# Autodesk Inventor assembly: FT7635M_Servo assembly_with T_BAR
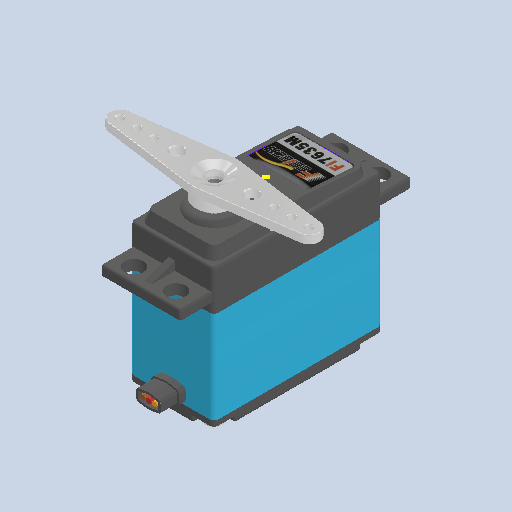
[picture p0: Inventor's stored thumbnail of the model, 512x512]
Saved by Autodesk Inventor 2025.3 (Build 293356000, 356)
## iProperties
Created: 2024-03-13
Part Number: FT7635M_Servo assembly_with T_BAR
Document SubType Name: Assembly
Designer: Eryk
Author: Eryk
## Documents named in this file (3)
- D:\Shooting Mechanism CAD\FT7635M_Servo assembly_with T_BAR.iam
- D:\Shooting Mechanism CAD\FT7635M_Servo assembly.iam
- D:\Shooting Mechanism CAD\Fleetech_FK-AP-4 (50 - 6) T-BAR.ipt
## Components (2 placed, 2 different names)
1. FT7635M_Servo assembly:1 [sub-assembly] — Mate:1, Mate:2
2. Fleetech_FK-AP-4 (50 - 6) T-BAR:1 — Mate:1, Mate:2
## Relationships (2: Mate 2)
- Mate:1: FT7635M_Servo assembly:1 ↔ Fleetech_FK-AP-4 (50 - 6) T-BAR:1
- Mate:2: FT7635M_Servo assembly:1 ↔ Fleetech_FK-AP-4 (50 - 6) T-BAR:1
